# Autodesk Inventor assembly: MAX Axel Hub
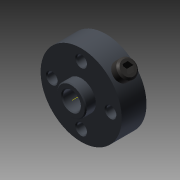
[picture p0: Inventor's stored thumbnail of the model, 180x180]
Saved by Autodesk Inventor 2015 (Build 190159000, 159)
## iProperties
Created: 2015-10-21
Part Number: MAX Axel Hub
Document SubType Name: Assembly
Designer: Mason
Author: Mason
## Documents named in this file (3)
- C:\Users\User\Documents\Inventor\Content Center Files\FTC\MAX Axel Hub.iam
- C:\Users\User\Documents\Inventor\Content Center Files\FTC\ASM parts DO NOT TOUCH\MAX Axel Hub .asm parts\MAX Axel Hub Collar.ipt
- C:\Users\User\Documents\Inventor\Content Center Files\FTC\ASM parts DO NOT TOUCH\MAX Axel Hub .asm parts\MAX Axel Hub Screw.ipt
## Components (2 placed, 2 different names)
1. MAX Axel Hub Collar:1 — Mate:1
2. MAX Axel Hub Screw:1 — Mate:1
## Relationships (1: Mate 1)
- Mate:1: MAX Axel Hub Collar:1 ↔ MAX Axel Hub Screw:1
